# Autodesk Inventor assembly: pole_gear_v2_with_clamp
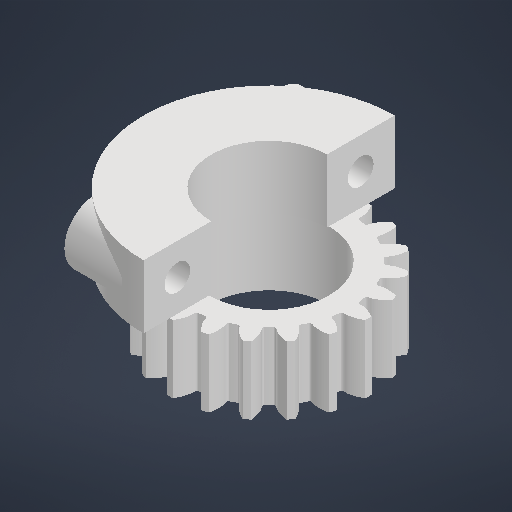
[picture p0: Inventor's stored thumbnail of the model, 512x512]
Saved by Autodesk Inventor 2026.2 (Build 302298000, 298)
## iProperties
Created: 2026-01-14
Part Number: pole_gear_v2_with_clamp
Document SubType Name: Assembly
Designer: User
Author: User
## Documents named in this file (3)
- C:\Users\User\Capstone\parts\turret assembly v2\pole_gear_v2_with_clamp.iam
- C:\Users\User\Capstone\parts\turret assembly v2\pole_gear_v2.ipt
- C:\Users\User\Capstone\parts\turret assembly v2\clamp_bolt.ipt
## Components (2 placed, 2 different names)
1. pole_gear_v2:1 — Mate:1, Mate:2
2. clamp_bolt:1 — Mate:1, Mate:2
## Relationships (2: Mate 2)
- Mate:1: pole_gear_v2:1 ↔ clamp_bolt:1
- Mate:2: pole_gear_v2:1 ↔ clamp_bolt:1
